# Autodesk Inventor assembly: VerticalSlides2.1
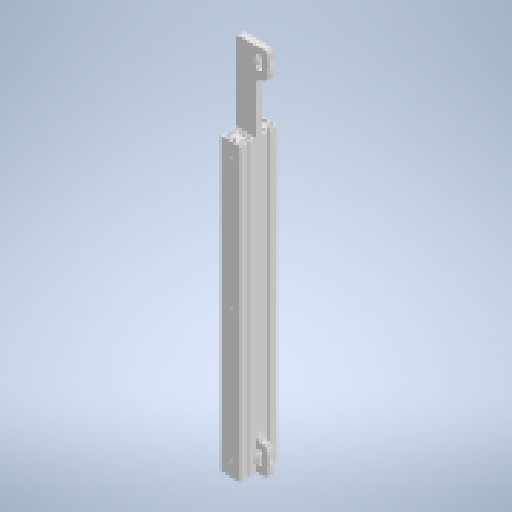
[picture p0: Inventor's stored thumbnail of the model, 512x512]
Saved by Autodesk Inventor 2023 (Build 270158000, 158)
## iProperties
Created: 2022-09-10
Part Number: VerticalSlides2.1
Document SubType Name: Assembly
Designer: deli
Author: deli
## Documents named in this file (5)
- C:\Users\deli\OneDrive - Eastside Preparatory School\FTC\8103-power-play\CAD\VerticalSlides2.1.iam
- C:\Users\deli\OneDrive - Eastside Preparatory School\FTC\8103-power-play\CAD\FTC-parts\KC-362-30.iam
- C:\Users\deli\OneDrive - Eastside Preparatory School\FTC\8103-power-play\CAD\FTC-parts\M3\hex_socket_button_head_M3x20.ipt
- C:\Users\deli\OneDrive - Eastside Preparatory School\FTC\8103-power-play\CAD\FTC-parts\LongRobotics\3x12x4mm-bearing.ipt
- C:\Users\deli\OneDrive - Eastside Preparatory School\FTC\8103-power-play\CAD\VerticalSlideMiddle2.1.ipt
## Components (7 placed, 4 different names)
1. KC-362-30:2 [sub-assembly] — Mate:49, Mate:50, Mate:51
2. KC-362-30:3 [sub-assembly] — Mate:46, Mate:47, Mate:48
3. hex_socket_button_head_M3x20:2 — Mate:55, Mate:56
4. hex_socket_button_head_M3x20:3 — Mate:52, Mate:53
5. 3x12x4mm-bearing:1 — Mate:54
6. 3x12x4mm-bearing:3 — Mate:57
7. VerticalSlideMiddle2.1:1 — Mate:46, Mate:47, Mate:48, Mate:49, Mate:50, Mate:51, Mate:52, Mate:53, Mate:54, Mate:55, Mate:56, Mate:57
## Relationships (14: Mate 14)
- [Mate]: hex_socket_button_head_M3x20:3 ↔ 3x12x4mm-bearing:1
- [Mate]: hex_socket_button_head_M3x20:2 ↔ 3x12x4mm-bearing:3
- Mate:46: KC-362-30:3 ↔ VerticalSlideMiddle2.1:1
- Mate:47: KC-362-30:3 ↔ VerticalSlideMiddle2.1:1
- Mate:48: KC-362-30:3 ↔ VerticalSlideMiddle2.1:1
- Mate:49: KC-362-30:2 ↔ VerticalSlideMiddle2.1:1
- Mate:50: KC-362-30:2 ↔ VerticalSlideMiddle2.1:1
- Mate:51: KC-362-30:2 ↔ VerticalSlideMiddle2.1:1
- Mate:52: hex_socket_button_head_M3x20:3 ↔ VerticalSlideMiddle2.1:1
- Mate:53: hex_socket_button_head_M3x20:3 ↔ VerticalSlideMiddle2.1:1
- Mate:54 (0.25 mm): 3x12x4mm-bearing:1 ↔ VerticalSlideMiddle2.1:1
- Mate:55: hex_socket_button_head_M3x20:2 ↔ VerticalSlideMiddle2.1:1
- Mate:56: hex_socket_button_head_M3x20:2 ↔ VerticalSlideMiddle2.1:1
- Mate:57 (0.25 mm): 3x12x4mm-bearing:3 ↔ VerticalSlideMiddle2.1:1
